# Autodesk Inventor assembly: Leg
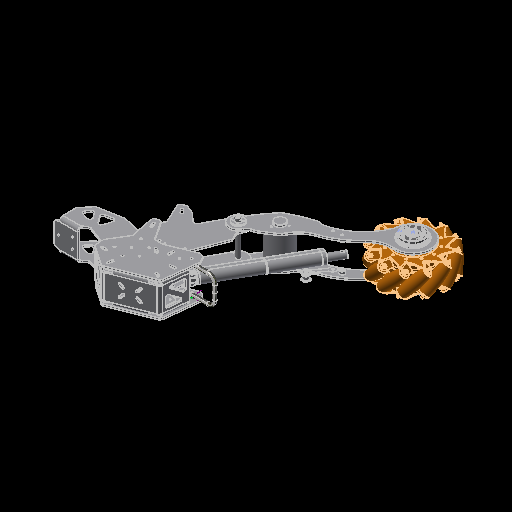
[picture p0: Inventor's stored thumbnail of the model, 512x512]
Saved by Autodesk Inventor 2025.2 (Build 292293000, 293)
## iProperties
Created: 2020-05-17
Part Number: Leg
Document SubType Name: Assembly
Designer: valer
_SolveAssemblyDoc: Frame Generator Solve Assembly
_Version: 15.0.0
Author: valer
## Documents named in this file (23)
- C:\Users\valer\Desktop\str1ker\cad\Leg.iam
- C:\Users\valer\Desktop\str1ker\cad\LegThigh.ipt
- C:\Users\valer\Desktop\str1ker\cad\LegShin.ipt
- C:\Users\valer\Desktop\str1ker\cad\LegHipSide.ipt
- C:\Users\valer\Desktop\str1ker\cad\LegHip.ipt
- C:\Users\valer\Desktop\str1ker\cad\LegHipFront.ipt
- C:\Users\valer\Desktop\str1ker\cad\external\2796N15_Omni-Directional Wheel.ipt
- C:\Users\valer\Desktop\str1ker\cad\external\MY6812-12VDC-120W-Motor.ipt
- C:\Users\valer\Desktop\str1ker\cad\external\SprocketMDEOOSKY-25H-47T.ipt
- C:\Users\valer\Desktop\str1ker\cad\LegHub.ipt
- C:\Users\valer\Desktop\str1ker\cad\external\6656K234_Ultra-Thin Ball Bearing.ipt
- C:\Users\valer\Desktop\str1ker\cad\LegInsideConnector.ipt
- C:\Users\valer\Desktop\str1ker\cad\external\FA-RMS-15-12-4.ipt
- C:\Users\valer\Desktop\str1ker\cad\external\FA-RMS-15-12-4-Piston.ipt
- C:\Users\valer\Desktop\str1ker\cad\external\LegPotentiometer\np32hs.iam
- C:\Users\valer\Desktop\str1ker\cad\LegHandleDesign.ipt
- C:\Users\valer\Desktop\str1ker\cad\LegKneeShaft.ipt
- C:\Users\valer\Desktop\str1ker\cad\external\Hub8mm.ipt
- C:\Users\valer\Desktop\str1ker\cad\external\2920-0001-0006 assembly.iam
- C:\Users\valer\Desktop\str1ker\cad\LegFrame\LegFrame.iam
- C:\Users\valer\Desktop\str1ker\cad\LegChainTensioner.iam
- C:\Users\valer\Desktop\str1ker\cad\external\WheelEncoder\am-4027 CIM_Coder_256_Encoder.iam
- C:\Users\valer\Desktop\str1ker\cad\external\WheelEncoder\am-4027 CIM_Coder_256_Magnet.iam
## Components (32 placed, 22 different names)
1. LegThigh:1 — Flush:1, Mate:1, Mate:4, Mate:163, Mate:173, Flush:145
2. LegHipSide:1 — Flush:1, Mate:1, Mate:4, Flush:140, Flush:141, Mate:152, Mate:153, Mate:154, Angle:2, Mate:161, Mate:168, Mate:171, Mate:180
3. LegThigh:2 — Mate:133, Flush:137, Mate:136, Mate:139, Mate:145, Mate:146
4. LegHipSide:2 — Mate:145, Mate:146, Mate:149, Flush:140, Flush:141, Mate:156, Mate:188
5. MY6812-12VDC-120W-Motor:1 — Mate:77, Mate:80, Mate:89, Mate:93, Flush:4, Flush:5, Mate:132, Mate:182, Flush:146
6. LegShin:3 — Mate:77, Mate:80, Mate:163, Mate:166, Mate:172, Mate:175, Mate:182, Mate:184, Mate:187, Mate:192, Mate:193
7. LegShin:4 — Mate:89, Mate:132, Mate:133, Mate:139, Mate:177, Mate:183, Mate:185, Mate:186
8. SprocketMDEOOSKY-25H-47T:1 — Flush:4, Mate:96, Mate:110, Flush:5, Mate:181, Mate:184
9. LegHub:1 — Mate:97, Mate:108, Mate:109, Mate:110, Mate:181
10. 2796N15_Omni-Directional Wheel:1 — Mate:96, Mate:97, Mate:102, Mate:103, Mate:104, Mate:105, Mate:106, Mate:107, Mate:108, Mate:109
11. 6656K234_Ultra-Thin Ball Bearing:1 — Mate:102, Mate:183
12. 6656K234_Ultra-Thin Ball Bearing:2 — Mate:103, Mate:104
13. LegHub:3 — Mate:105, Mate:106, Mate:107, Mate:195, Mate:196, Mate:197
14. FA-RMS-15-12-4:1 — Mate:125, Mate:149, Mate:167, Mate:189, Mate:191
15. np32hs:1 [sub-assembly] — Flush:137, Mate:136, Angle:4
16. LegHandleDesign:1 — Flush:143, Mate:170, Mate:171
17. LegKneeShaft:1 — Mate:172, Mate:173, Mate:174, Mate:176, Angle:4, Flush:144, Flush:145
18. LegHip:1 — Mate:152, Mate:153, Mate:154, Mate:155, Mate:157, Mate:164, Flush:142, Mate:178
19. LegInsideConnector:5 — Mate:155, Mate:156, Mate:157, Mate:162, Mate:179
20. LegHipFront:1 — Angle:2, Mate:161, Mate:162, Mate:165
21. FA-RMS-15-12-4-Piston:1 — Mate:166, Mate:167
22. Hub8mm:1 — Mate:174, Mate:175, Flush:144
23. Hub8mm:2 — Mate:176, Mate:177
24. LegInsideConnector:6 — Mate:178, Mate:179, Mate:180
25. 2920-0001-0006 assembly:1 [sub-assembly] — Mate:185, Mate:186
26. 2920-0001-0006 assembly:2 [sub-assembly] — Mate:187, Mate:192
27. 2920-0001-0006 assembly:3 [sub-assembly] — Mate:188, Mate:189
28. 2920-0001-0006 assembly:4 [sub-assembly] — Mate:191
29. LegFrame:1 [sub-assembly]
30. LegChainTensioner:1 [sub-assembly] — Flush:146, Mate:193
31. am-4027 CIM_Coder_256_Encoder:1 [sub-assembly] — Mate:196, Mate:198
32. am-4027 CIM_Coder_256_Magnet:1 [sub-assembly] — Mate:195, Mate:197, Mate:198
## Relationships (80: Mate 66, Flush 11, Angle 3)
- Flush:1 (-5.08 mm): LegThigh:1 ↔ LegHipSide:1
- Mate:1: LegThigh:1 ↔ LegHipSide:1
- Mate:4: LegThigh:1 ↔ LegHipSide:1
- Mate:77: MY6812-12VDC-120W-Motor:1 ↔ LegShin:3
- Mate:80: MY6812-12VDC-120W-Motor:1 ↔ LegShin:3
- Mate:89: MY6812-12VDC-120W-Motor:1 ↔ LegShin:4
- Mate:93: MY6812-12VDC-120W-Motor:1
- Flush:4: MY6812-12VDC-120W-Motor:1 ↔ SprocketMDEOOSKY-25H-47T:1
- Mate:96: SprocketMDEOOSKY-25H-47T:1 ↔ 2796N15_Omni-Directional Wheel:1
- Mate:97: LegHub:1 ↔ 2796N15_Omni-Directional Wheel:1
- Mate:102: 2796N15_Omni-Directional Wheel:1 ↔ 6656K234_Ultra-Thin Ball Bearing:1
- Mate:103: 2796N15_Omni-Directional Wheel:1 ↔ 6656K234_Ultra-Thin Ball Bearing:2
- Mate:104: 2796N15_Omni-Directional Wheel:1 ↔ 6656K234_Ultra-Thin Ball Bearing:2
- Mate:105: 2796N15_Omni-Directional Wheel:1 ↔ LegHub:3
- Mate:106: 2796N15_Omni-Directional Wheel:1 ↔ LegHub:3
- Mate:107: 2796N15_Omni-Directional Wheel:1 ↔ LegHub:3
- Mate:108: LegHub:1 ↔ 2796N15_Omni-Directional Wheel:1
- Mate:109: LegHub:1 ↔ 2796N15_Omni-Directional Wheel:1
- Mate:110: SprocketMDEOOSKY-25H-47T:1 ↔ LegHub:1
- Flush:5: MY6812-12VDC-120W-Motor:1 ↔ SprocketMDEOOSKY-25H-47T:1
- Mate:125: FA-RMS-15-12-4:1
- Mate:132: MY6812-12VDC-120W-Motor:1 ↔ LegShin:4
- Mate:133: LegThigh:2 ↔ LegShin:4
- Flush:137: LegThigh:2 ↔ np32hs:1
- Mate:136: LegThigh:2 ↔ np32hs:1
- Mate:139: LegThigh:2 ↔ LegShin:4
- Mate:145: LegThigh:2 ↔ LegHipSide:2
- Mate:146: LegThigh:2 ↔ LegHipSide:2
- Mate:149: LegHipSide:2 ↔ FA-RMS-15-12-4:1
- Flush:140: LegHipSide:1 ↔ LegHipSide:2
- Flush:141: LegHipSide:1 ↔ LegHipSide:2
- Mate:152: LegHipSide:1 ↔ LegHip:1
- Mate:153: LegHipSide:1 ↔ LegHip:1
- Mate:154: LegHipSide:1 ↔ LegHip:1
- Mate:155: LegHip:1 ↔ LegInsideConnector:5
- Mate:156: LegHipSide:2 ↔ LegInsideConnector:5
- Mate:157: LegHip:1 ↔ LegInsideConnector:5
- Angle:2 (0 deg): LegHipSide:1 ↔ LegHipFront:1
- Mate:161: LegHipSide:1 ↔ LegHipFront:1
- Mate:162: LegInsideConnector:5 ↔ LegHipFront:1
- Mate:163: LegThigh:1 ↔ LegShin:3
- Mate:164: LegHip:1
- Mate:165: LegHipFront:1
- Flush:142: LegHip:1
- Mate:166: LegShin:3 ↔ FA-RMS-15-12-4-Piston:1
- Mate:167: FA-RMS-15-12-4:1 ↔ FA-RMS-15-12-4-Piston:1
- Mate:168: LegHipSide:1
- Angle:3 (0 deg)
- Flush:143: LegHandleDesign:1
- Mate:170: LegHandleDesign:1
- Mate:171: LegHipSide:1 ↔ LegHandleDesign:1
- Mate:172: LegShin:3 ↔ LegKneeShaft:1
- Mate:173: LegThigh:1 ↔ LegKneeShaft:1
- Mate:174: LegKneeShaft:1 ↔ Hub8mm:1
- Mate:175: LegShin:3 ↔ Hub8mm:1
- Mate:176: LegKneeShaft:1 ↔ Hub8mm:2
- Mate:177: LegShin:4 ↔ Hub8mm:2
- Angle:4 (180 deg): np32hs:1 ↔ LegKneeShaft:1
- Flush:144: LegKneeShaft:1 ↔ Hub8mm:1
- Flush:145 (0.5 mm): LegThigh:1 ↔ LegKneeShaft:1
- Mate:178: LegHip:1 ↔ LegInsideConnector:6
- Mate:179: LegInsideConnector:5 ↔ LegInsideConnector:6
- Mate:180: LegHipSide:1 ↔ LegInsideConnector:6
- Mate:181: SprocketMDEOOSKY-25H-47T:1 ↔ LegHub:1
- Mate:182: MY6812-12VDC-120W-Motor:1 ↔ LegShin:3
- Mate:183: LegShin:4 ↔ 6656K234_Ultra-Thin Ball Bearing:1
- Mate:184: LegShin:3 ↔ SprocketMDEOOSKY-25H-47T:1
- Mate:185: LegShin:4 ↔ 2920-0001-0006 assembly:1
- Mate:186: LegShin:4 ↔ 2920-0001-0006 assembly:1
- Mate:187: LegShin:3 ↔ 2920-0001-0006 assembly:2
- Mate:188: LegHipSide:2 ↔ 2920-0001-0006 assembly:3
- Mate:189: FA-RMS-15-12-4:1 ↔ 2920-0001-0006 assembly:3
- Mate:191: FA-RMS-15-12-4:1 ↔ 2920-0001-0006 assembly:4
- Mate:192: LegShin:3 ↔ 2920-0001-0006 assembly:2
- Flush:146: MY6812-12VDC-120W-Motor:1 ↔ LegChainTensioner:1
- Mate:193: LegShin:3 ↔ LegChainTensioner:1
- Mate:195: LegHub:3 ↔ am-4027 CIM_Coder_256_Magnet:1
- Mate:196: LegHub:3 ↔ am-4027 CIM_Coder_256_Encoder:1
- Mate:197: LegHub:3 ↔ am-4027 CIM_Coder_256_Magnet:1
- Mate:198: am-4027 CIM_Coder_256_Encoder:1 ↔ am-4027 CIM_Coder_256_Magnet:1
